# Autodesk Inventor assembly: Assembly1
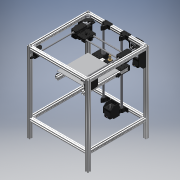
[picture p0: Inventor's stored thumbnail of the model, 180x180]
Saved by Autodesk Inventor 2018 (Build 220112000, 112)
## iProperties
Created: 2018-05-23
Part Number: Assembly1
Document SubType Name: Assembly
Designer: Z. Deniz
Author: Z. Deniz
## Documents named in this file (20)
- C:\Users\zdeni\Desktop\my3D\3D_Model_v2\main_frame.iam
- C:\Users\zdeni\Desktop\my3D\3D_Model_v2\parçalar\2020 Extrusion 550mm.ipt
- C:\Users\zdeni\Desktop\my3D\3D_Model_v2\parçalar\2020 Extrusion 380mm.ipt
- C:\Users\zdeni\Desktop\my3D\3D_Model_v2\parçalar\90 angle.ipt
- C:\Users\zdeni\Desktop\my3D\3D_Model_v2\montajlar\bed_assembly.iam
- C:\Users\zdeni\Desktop\my3D\3D_Model_v2\parçalar\450mm mil.ipt
- C:\Users\zdeni\Desktop\my3D\3D_Model_v2\parçalar\z_rod_holder.ipt
- C:\Users\zdeni\Desktop\my3D\3D_Model_v2\parçalar\380mm mil.ipt
- C:\Users\zdeni\Desktop\my3D\3D_Model_v2\parçalar\320mm mil.ipt
- C:\Users\zdeni\Desktop\my3D\3D_Model_v2\parçalar\nema17_holder_left.ipt
- C:\Users\zdeni\Desktop\my3D\3D_Model_v2\parçalar\nema17_holder_right.ipt
- C:\Users\zdeni\Desktop\my3D\3D_Model_v2\parçalar\modeller\256517HM19-2004S.ipt
- C:\Users\zdeni\Desktop\my3D\3D_Model_v2\parçalar\front_belt-rod_holder_left_v2.ipt
- C:\Users\zdeni\Desktop\my3D\3D_Model_v2\parçalar\front_belt-rod_holder_right_v2.ipt
- C:\Users\zdeni\Desktop\my3D\3D_Model_v2\parçalar\support.ipt
- C:\Users\zdeni\Desktop\my3D\3D_Model_v2\parçalar\nema17_holder_z.ipt
- C:\Users\zdeni\Desktop\my3D\3D_Model_v2\montajlar\xy_assembly.iam
- C:\Users\zdeni\Desktop\my3D\3D_Model_v2\parçalar\modeller\GT2_32teeth_10bore.ipt
- C:\Users\zdeni\Desktop\my3D\3D_Model_v2\montajlar\hotend_assembly.iam
- C:\Users\zdeni\Desktop\my3D\3D_Model_v2\parçalar\extr_motor_holder.ipt
## Components (63 placed, 19 different names)
1. 2020 Extrusion 550mm:1 — Mate:5, Flush:8, Mate:6, Flush:9, Mate:9, Flush:18, Mate:12, Mate:57, Flush:61, Mate:71, Mate:83, Mate:86, Mate:91, Mate:105, Flush:67
2. 2020 Extrusion 550mm:2 — Mate:7, Flush:11, Flush:14, Flush:22, Flush:23, Flush:24, Flush:25, Mate:30, Flush:45, Mate:36, Mate:51, Mate:74, Mate:77, Mate:82, Flush:68
3. 2020 Extrusion 550mm:3 — Mate:1, Flush:1, Mate:4, Flush:6, Flush:19, Mate:10, Mate:60, Flush:56, Mate:94, Mate:96, Mate:115, Flush:66
4. 2020 Extrusion 550mm:4 — Mate:3, Flush:2, Mate:8, Flush:20, Flush:21, Mate:11, Mate:21, Mate:54, Flush:53, Mate:64, Flush:58, Mate:99, Mate:103
5. 2020 Extrusion 380mm:1 — Mate:9, Flush:18, Flush:19, Mate:14, Flush:38, Mate:15
6. 2020 Extrusion 380mm:2 — Mate:6, Flush:9, Mate:7, Flush:11, Flush:15, Flush:17, Flush:42, Flush:43, Tangent:3, Tangent:4, Mate:22, Mate:23, Mate:24, Mate:25, Mate:49, Mate:50, Flush:51, Mate:56, Flush:54, Mate:59, Mate:76, Mate:79, Mate:80, Mate:85, Mate:88, Mate:89, Flush:67, Flush:68, Mate:127, Flush:72
7. 2020 Extrusion 380mm:3 — Flush:5, Mate:4, Flush:6, Mate:5, Flush:8, Flush:17, Mate:33, Mate:34, Mate:58, Flush:55, Mate:62, Flush:57, Mate:70, Mate:114, Flush:66
8. 2020 Extrusion 380mm:4 — Mate:10, Flush:20, Flush:21, Mate:13, Mate:20, Flush:41
9. 2020 Extrusion 380mm:5 — Mate:1, Flush:1, Mate:3, Flush:2, Flush:5, Mate:31, Mate:32, Mate:52, Flush:52, Mate:55, Mate:61, Mate:63, Mate:93, Mate:97, Mate:100, Mate:102
10. 2020 Extrusion 380mm:6 — Mate:11, Flush:22, Flush:23, Mate:17, Flush:40, Mate:19
11. 2020 Extrusion 380mm:7 — Mate:8, Flush:14, Flush:15, Tangent:5, Mate:35, Mate:48, Flush:50, Mate:53, Angle:1
12. 2020 Extrusion 380mm:8 — Mate:12, Flush:24, Flush:25, Mate:16, Flush:39, Mate:18, Mate:26, Mate:27, Mate:28, Mate:29, Mate:104, Flush:62, Mate:106, Mate:108, Mate:110
13. 90 angle:1 — Mate:13, Mate:14, Flush:38
14. 90 angle:2 — Mate:15, Mate:16, Flush:39
15. 90 angle:3 — Mate:19, Mate:20, Flush:41
16. 90 angle:4 — Mate:17, Mate:18, Flush:40
17. bed_assembly:1 [sub-assembly] — Tangent:1, Tangent:2, Flush:44
18. 450mm mil:1 — Flush:42, Tangent:1, Tangent:3, Tangent:5, Tangent:7, Tangent:8
19. 450mm mil:2 — Flush:43, Tangent:2, Tangent:4, Flush:44, Tangent:6, Tangent:9
20. z_rod_holder:1 — Mate:26, Tangent:8, Mate:27
21. z_rod_holder:2 — Mate:24, Tangent:7, Mate:25
22. z_rod_holder:3 — Mate:28, Tangent:9, Mate:29
23. z_rod_holder:4 — Mate:22, Tangent:6, Mate:23
24. 380mm mil:1 — Mate:31, Tangent:26, Tangent:30, Mate:116
25. 380mm mil:2 — Mate:32, Tangent:10, Tangent:19, Mate:113
26. 320mm mil:1 — Mate:34, Mate:119, Mate:125, Mate:126
27. 320mm mil:2 — Mate:33, Tangent:32, Angle:1, Angle:2, Mate:120, Mate:123, Mate:124
28. nema17_holder_left:1 — Mate:35, Flush:45, Mate:36, Tangent:10, Mate:42, Tangent:14, Tangent:15, Mate:75, Mate:78, Mate:81
29. nema17_holder_right:1 — Mate:69, Tangent:24, Tangent:25, Tangent:26, Flush:61, Mate:70, Mate:71, Mate:84, Mate:87, Mate:90, Mate:130
30. 256517HM19-2004S:1 — Mate:42, Tangent:14, Tangent:15, Insert:1
31. 256517HM19-2004S:2 — Mate:69, Tangent:24, Tangent:25, Insert:2
32. 90 angle:5 — Mate:48, Mate:49, Flush:50
33. 90 angle:6 — Mate:50, Mate:51, Flush:51
34. 90 angle:7 — Mate:54, Mate:55, Flush:53
35. 90 angle:8 — Mate:52, Mate:53, Flush:52
36. 90 angle:9 — Mate:62, Mate:63, Flush:57
37. 90 angle:10 — Mate:60, Mate:61, Flush:56
38. 90 angle:11 — Mate:56, Mate:57, Flush:54
39. 90 angle:12 — Mate:58, Mate:59, Flush:55
40. front_belt-rod_holder_left_v2:1 — Mate:64, Flush:58, Tangent:19, Mate:98, Mate:101, Mate:121
41. front_belt-rod_holder_right_v2:1 — Tangent:30, Mate:114, Mate:115
42. support:1 — Mate:86, Mate:87, Mate:88
43. support:2 — Mate:101, Mate:102, Mate:103
44. support:3 — Mate:83, Mate:84, Mate:85
45. support:4 — Mate:80, Mate:81, Mate:82
46. support:6 — Mate:98, Mate:99, Mate:100
47. support:7 — Mate:74, Mate:75, Mate:76
48. support:8 — Mate:77, Mate:78, Mate:79
49. support:9 — Mate:93, Mate:94
50. support:10 — Mate:96, Mate:97
51. support:11 — Mate:89, Mate:90, Mate:91
52. nema17_holder_z:1 — Mate:104, Flush:62, Mate:105, Mate:107, Flush:63, Mate:109, Flush:64, Mate:111, Flush:65, Tangent:28, Mate:112, Tangent:29, Mate:118
53. support:12 — Mate:106, Mate:107, Flush:63
54. support:13 — Mate:108, Mate:109, Flush:64
55. support:14 — Mate:110, Mate:111, Flush:65
56. 256517HM19-2004S:3 — Tangent:28, Mate:112, Tangent:29, Mate:118
57. xy_assembly:1 [sub-assembly] — Mate:113, Tangent:32, Angle:2, Mate:121, Mate:122, Mate:123, Mate:125
58. xy_assembly:2 [sub-assembly] — Mate:116, Mate:124, Mate:126
59. GT2_32teeth_10bore:1 — Insert:1
60. GT2_32teeth_10bore:2 — Insert:2
61. hotend_assembly:1 [sub-assembly] — Mate:119, Mate:120, Mate:122
62. extr_motor_holder:1 — Mate:127, Flush:70, Flush:71, Mate:129, Flush:72
63. 256517HM19-2004S:4 — Flush:70, Flush:71, Mate:129, Mate:130
## Relationships (179: Mate 109, Flush 46, Tangent 20, Angle 2, Insert 2)
- Mate:1: 2020 Extrusion 550mm:3 ↔ 2020 Extrusion 380mm:5
- Flush:1: 2020 Extrusion 550mm:3 ↔ 2020 Extrusion 380mm:5
- Mate:3: 2020 Extrusion 550mm:4 ↔ 2020 Extrusion 380mm:5
- Flush:2: 2020 Extrusion 550mm:4 ↔ 2020 Extrusion 380mm:5
- Flush:5: 2020 Extrusion 380mm:3 ↔ 2020 Extrusion 380mm:5
- Mate:4: 2020 Extrusion 550mm:3 ↔ 2020 Extrusion 380mm:3
- Flush:6: 2020 Extrusion 550mm:3 ↔ 2020 Extrusion 380mm:3
- Mate:5: 2020 Extrusion 550mm:1 ↔ 2020 Extrusion 380mm:3
- Flush:8: 2020 Extrusion 550mm:1 ↔ 2020 Extrusion 380mm:3
- Mate:6: 2020 Extrusion 550mm:1 ↔ 2020 Extrusion 380mm:2
- Flush:9: 2020 Extrusion 550mm:1 ↔ 2020 Extrusion 380mm:2
- Mate:7: 2020 Extrusion 550mm:2 ↔ 2020 Extrusion 380mm:2
- Flush:11: 2020 Extrusion 550mm:2 ↔ 2020 Extrusion 380mm:2
- Mate:8: 2020 Extrusion 550mm:4 ↔ 2020 Extrusion 380mm:7
- Flush:14: 2020 Extrusion 550mm:2 ↔ 2020 Extrusion 380mm:7
- Flush:15: 2020 Extrusion 380mm:2 ↔ 2020 Extrusion 380mm:7
- Flush:17: 2020 Extrusion 380mm:2 ↔ 2020 Extrusion 380mm:3
- Mate:9: 2020 Extrusion 550mm:1 ↔ 2020 Extrusion 380mm:1
- Flush:18: 2020 Extrusion 550mm:1 ↔ 2020 Extrusion 380mm:1
- Flush:19 (105 mm): 2020 Extrusion 550mm:3 ↔ 2020 Extrusion 380mm:1
- Mate:10: 2020 Extrusion 550mm:3 ↔ 2020 Extrusion 380mm:4
- Flush:20: 2020 Extrusion 550mm:4 ↔ 2020 Extrusion 380mm:4
- Flush:21 (105 mm): 2020 Extrusion 550mm:4 ↔ 2020 Extrusion 380mm:4
- Mate:11: 2020 Extrusion 550mm:4 ↔ 2020 Extrusion 380mm:6
- Flush:22: 2020 Extrusion 550mm:2 ↔ 2020 Extrusion 380mm:6
- Flush:23 (105 mm): 2020 Extrusion 550mm:2 ↔ 2020 Extrusion 380mm:6
- Mate:12: 2020 Extrusion 550mm:1 ↔ 2020 Extrusion 380mm:8
- Flush:24: 2020 Extrusion 550mm:2 ↔ 2020 Extrusion 380mm:8
- Flush:25 (105 mm): 2020 Extrusion 550mm:2 ↔ 2020 Extrusion 380mm:8
- Mate:13: 2020 Extrusion 380mm:4 ↔ 90 angle:1
- Mate:14: 2020 Extrusion 380mm:1 ↔ 90 angle:1
- Flush:38 (1.5 mm): 2020 Extrusion 380mm:1 ↔ 90 angle:1
- Mate:15: 2020 Extrusion 380mm:1 ↔ 90 angle:2
- Mate:16: 2020 Extrusion 380mm:8 ↔ 90 angle:2
- Flush:39 (1.5 mm): 2020 Extrusion 380mm:8 ↔ 90 angle:2
- Mate:17: 2020 Extrusion 380mm:6 ↔ 90 angle:4
- Mate:18: 2020 Extrusion 380mm:8 ↔ 90 angle:4
- Flush:40 (1.5 mm): 2020 Extrusion 380mm:6 ↔ 90 angle:4
- Mate:19: 2020 Extrusion 380mm:6 ↔ 90 angle:3
- Mate:20: 2020 Extrusion 380mm:4 ↔ 90 angle:3
- Flush:41 (1.5 mm): 2020 Extrusion 380mm:4 ↔ 90 angle:3
- Flush:42: 2020 Extrusion 380mm:2 ↔ 450mm mil:1
- Flush:43: 2020 Extrusion 380mm:2 ↔ 450mm mil:2
- Tangent:1: bed_assembly:1 ↔ 450mm mil:1
- Tangent:2: bed_assembly:1 ↔ 450mm mil:2
- Tangent:3 (15 mm): 2020 Extrusion 380mm:2 ↔ 450mm mil:1
- Tangent:4 (15 mm): 2020 Extrusion 380mm:2 ↔ 450mm mil:2
- Flush:44 (150 mm): bed_assembly:1 ↔ 450mm mil:2
- Tangent:5 (121.5 mm): 2020 Extrusion 380mm:7 ↔ 450mm mil:1
- Mate:21: 2020 Extrusion 550mm:4
- Mate:22: 2020 Extrusion 380mm:2 ↔ z_rod_holder:4
- Tangent:6: 450mm mil:2 ↔ z_rod_holder:4
- Mate:23: 2020 Extrusion 380mm:2 ↔ z_rod_holder:4
- Mate:24: 2020 Extrusion 380mm:2 ↔ z_rod_holder:2
- Tangent:7: 450mm mil:1 ↔ z_rod_holder:2
- Mate:25: 2020 Extrusion 380mm:2 ↔ z_rod_holder:2
- Mate:26: 2020 Extrusion 380mm:8 ↔ z_rod_holder:1
- Tangent:8: 450mm mil:1 ↔ z_rod_holder:1
- Mate:27: 2020 Extrusion 380mm:8 ↔ z_rod_holder:1
- Mate:28: 2020 Extrusion 380mm:8 ↔ z_rod_holder:3
- Tangent:9: 450mm mil:2 ↔ z_rod_holder:3
- Mate:29: 2020 Extrusion 380mm:8 ↔ z_rod_holder:3
- Mate:30: 2020 Extrusion 550mm:2
- Mate:31: 2020 Extrusion 380mm:5 ↔ 380mm mil:1
- Mate:32: 2020 Extrusion 380mm:5 ↔ 380mm mil:2
- Mate:33 (30 mm): 2020 Extrusion 380mm:3 ↔ 320mm mil:2
- Mate:34 (30 mm): 2020 Extrusion 380mm:3 ↔ 320mm mil:1
- Mate:35: 2020 Extrusion 380mm:7 ↔ nema17_holder_left:1
- Flush:45: 2020 Extrusion 550mm:2 ↔ nema17_holder_left:1
- Mate:36: 2020 Extrusion 550mm:2 ↔ nema17_holder_left:1
- Tangent:10: 380mm mil:2 ↔ nema17_holder_left:1
- Mate:42: nema17_holder_left:1 ↔ 256517HM19-2004S:1
- Tangent:14: nema17_holder_left:1 ↔ 256517HM19-2004S:1
- Tangent:15: nema17_holder_left:1 ↔ 256517HM19-2004S:1
- Mate:48: 2020 Extrusion 380mm:7 ↔ 90 angle:5
- Mate:49: 2020 Extrusion 380mm:2 ↔ 90 angle:5
- Flush:50 (1.5 mm): 2020 Extrusion 380mm:7 ↔ 90 angle:5
- Mate:50: 2020 Extrusion 380mm:2 ↔ 90 angle:6
- Mate:51: 2020 Extrusion 550mm:2 ↔ 90 angle:6
- Flush:51 (1.5 mm): 2020 Extrusion 380mm:2 ↔ 90 angle:6
- Mate:52: 2020 Extrusion 380mm:5 ↔ 90 angle:8
- Mate:53: 2020 Extrusion 380mm:7 ↔ 90 angle:8
- Flush:52 (1.5 mm): 2020 Extrusion 380mm:5 ↔ 90 angle:8
- Mate:54: 2020 Extrusion 550mm:4 ↔ 90 angle:7
- Mate:55: 2020 Extrusion 380mm:5 ↔ 90 angle:7
- Flush:53 (1.5 mm): 2020 Extrusion 550mm:4 ↔ 90 angle:7
- Mate:56: 2020 Extrusion 380mm:2 ↔ 90 angle:11
- Mate:57: 2020 Extrusion 550mm:1 ↔ 90 angle:11
- Flush:54 (1.5 mm): 2020 Extrusion 380mm:2 ↔ 90 angle:11
- Mate:58: 2020 Extrusion 380mm:3 ↔ 90 angle:12
- Mate:59: 2020 Extrusion 380mm:2 ↔ 90 angle:12
- Flush:55 (1.5 mm): 2020 Extrusion 380mm:3 ↔ 90 angle:12
- Mate:60: 2020 Extrusion 550mm:3 ↔ 90 angle:10
- Mate:61: 2020 Extrusion 380mm:5 ↔ 90 angle:10
- Flush:56 (1.5 mm): 2020 Extrusion 550mm:3 ↔ 90 angle:10
- Mate:62: 2020 Extrusion 380mm:3 ↔ 90 angle:9
- Mate:63: 2020 Extrusion 380mm:5 ↔ 90 angle:9
- Flush:57 (1.5 mm): 2020 Extrusion 380mm:3 ↔ 90 angle:9
- Mate:64: 2020 Extrusion 550mm:4 ↔ front_belt-rod_holder_left_v2:1
- Flush:58: 2020 Extrusion 550mm:4 ↔ front_belt-rod_holder_left_v2:1
- Tangent:19: 380mm mil:2 ↔ front_belt-rod_holder_left_v2:1
- Mate:69: nema17_holder_right:1 ↔ 256517HM19-2004S:2
- Tangent:24: nema17_holder_right:1 ↔ 256517HM19-2004S:2
- Tangent:25: nema17_holder_right:1 ↔ 256517HM19-2004S:2
- Tangent:26: 380mm mil:1 ↔ nema17_holder_right:1
- Flush:61: 2020 Extrusion 550mm:1 ↔ nema17_holder_right:1
- Mate:70: 2020 Extrusion 380mm:3 ↔ nema17_holder_right:1
- Mate:71: 2020 Extrusion 550mm:1 ↔ nema17_holder_right:1
- Mate:74: 2020 Extrusion 550mm:2 ↔ support:7
- Mate:75: nema17_holder_left:1 ↔ support:7
- Mate:76 (60 mm): 2020 Extrusion 380mm:2 ↔ support:7
- Mate:77: 2020 Extrusion 550mm:2 ↔ support:8
- Mate:78: nema17_holder_left:1 ↔ support:8
- Mate:79 (30 mm): 2020 Extrusion 380mm:2 ↔ support:8
- Mate:80: 2020 Extrusion 380mm:2 ↔ support:4
- Mate:81: nema17_holder_left:1 ↔ support:4
- Mate:82 (20 mm): 2020 Extrusion 550mm:2 ↔ support:4
- Mate:83: 2020 Extrusion 550mm:1 ↔ support:3
- Mate:84: nema17_holder_right:1 ↔ support:3
- Mate:85 (60 mm): 2020 Extrusion 380mm:2 ↔ support:3
- Mate:86: 2020 Extrusion 550mm:1 ↔ support:1
- Mate:87: nema17_holder_right:1 ↔ support:1
- Mate:88 (30 mm): 2020 Extrusion 380mm:2 ↔ support:1
- Mate:89: 2020 Extrusion 380mm:2 ↔ support:11
- Mate:90: nema17_holder_right:1 ↔ support:11
- Mate:91 (20 mm): 2020 Extrusion 550mm:1 ↔ support:11
- Mate:93: 2020 Extrusion 380mm:5 ↔ support:9
- Mate:94 (20 mm): 2020 Extrusion 550mm:3 ↔ support:9
- Mate:96: 2020 Extrusion 550mm:3 ↔ support:10
- Mate:97 (40 mm): 2020 Extrusion 380mm:5 ↔ support:10
- Mate:98: front_belt-rod_holder_left_v2:1 ↔ support:6
- Mate:99: 2020 Extrusion 550mm:4 ↔ support:6
- Mate:100 (40 mm): 2020 Extrusion 380mm:5 ↔ support:6
- Mate:101: front_belt-rod_holder_left_v2:1 ↔ support:2
- Mate:102: 2020 Extrusion 380mm:5 ↔ support:2
- Mate:103 (20 mm): 2020 Extrusion 550mm:4 ↔ support:2
- Mate:104: 2020 Extrusion 380mm:8 ↔ nema17_holder_z:1
- Flush:62: 2020 Extrusion 380mm:8 ↔ nema17_holder_z:1
- Mate:105 (162.5 mm): 2020 Extrusion 550mm:1 ↔ nema17_holder_z:1
- Mate:106: 2020 Extrusion 380mm:8 ↔ support:12
- Mate:107: nema17_holder_z:1 ↔ support:12
- Flush:63: nema17_holder_z:1 ↔ support:12
- Mate:108: 2020 Extrusion 380mm:8 ↔ support:13
- Mate:109: nema17_holder_z:1 ↔ support:13
- Flush:64: nema17_holder_z:1 ↔ support:13
- Mate:110: 2020 Extrusion 380mm:8 ↔ support:14
- Mate:111: nema17_holder_z:1 ↔ support:14
- Flush:65 (22.5 mm): nema17_holder_z:1 ↔ support:14
- Tangent:28: nema17_holder_z:1 ↔ 256517HM19-2004S:3
- Mate:112: nema17_holder_z:1 ↔ 256517HM19-2004S:3
- Tangent:29: nema17_holder_z:1 ↔ 256517HM19-2004S:3
- Mate:113: 380mm mil:2 ↔ xy_assembly:1
- Tangent:30: 380mm mil:1 ↔ front_belt-rod_holder_right_v2:1
- Mate:114: 2020 Extrusion 380mm:3 ↔ front_belt-rod_holder_right_v2:1
- Mate:115: 2020 Extrusion 550mm:3 ↔ front_belt-rod_holder_right_v2:1
- Tangent:32: 320mm mil:2 ↔ xy_assembly:1
- Mate:116: 380mm mil:1 ↔ xy_assembly:2
- Angle:1 (0 deg): 2020 Extrusion 380mm:7 ↔ 320mm mil:2
- Angle:2 (0 deg): 320mm mil:2 ↔ xy_assembly:1
- Mate:118 (1.5 mm): nema17_holder_z:1 ↔ 256517HM19-2004S:3
- Insert:1 (16.5 mm): 256517HM19-2004S:1 ↔ GT2_32teeth_10bore:1
- Insert:2 (-3.5 mm): 256517HM19-2004S:2 ↔ GT2_32teeth_10bore:2
- Mate:119: 320mm mil:1 ↔ hotend_assembly:1
- Mate:120: 320mm mil:2 ↔ hotend_assembly:1
- Mate:121: front_belt-rod_holder_left_v2:1 ↔ xy_assembly:1
- Mate:122: xy_assembly:1 ↔ hotend_assembly:1
- Flush:66: 2020 Extrusion 550mm:3 ↔ 2020 Extrusion 380mm:3
- Flush:67: 2020 Extrusion 550mm:1 ↔ 2020 Extrusion 380mm:2
- Flush:68: 2020 Extrusion 550mm:2 ↔ 2020 Extrusion 380mm:2
- Mate:123: 320mm mil:2 ↔ xy_assembly:1
- Mate:124: 320mm mil:2 ↔ xy_assembly:2
- Mate:125: 320mm mil:1 ↔ xy_assembly:1
- Mate:126: 320mm mil:1 ↔ xy_assembly:2
- Mate:127: 2020 Extrusion 380mm:2 ↔ extr_motor_holder:1
- Flush:70: extr_motor_holder:1 ↔ 256517HM19-2004S:4
- Flush:71: extr_motor_holder:1 ↔ 256517HM19-2004S:4
- Mate:129: extr_motor_holder:1 ↔ 256517HM19-2004S:4
- Flush:72: 2020 Extrusion 380mm:2 ↔ extr_motor_holder:1
- Mate:130: nema17_holder_right:1 ↔ 256517HM19-2004S:4
## Named parameters: corner_d = 1 mm, base_h = 105 mm, bed_rod_d = 15 mm, bed_h = 150 mm
